# Autodesk Inventor assembly: ASM_Micron_Exploded
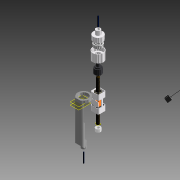
[picture p0: Inventor's stored thumbnail of the model, 180x180]
Saved by Autodesk Inventor 2011 SP2 (Build 150309200, 309)
## iProperties
Created: 2013-06-24
Part Number: ASM_Micron_Exploded
Document SubType Name: Assembly
Designer: sungwook
Author: sungwook
## Documents named in this file (10)
- C:\Users\sungwook\Documents\Inventor\Micron22_top_adj_02082013\06242013_FigGen\ASM_Micron_Motor_Exploded.iam
- C:\Users\sungwook\Documents\Inventor\Micron22_top_adj_02082013\Parts\Motor Units\MU_Motor_Asm_Frame_new3.ipt
- C:\Users\sungwook\Documents\Inventor\Micron22_top_adj_02082013\Parts\Motor Units\Squiggle\MU_SQ_Motor_Base.iam
- C:\Users\sungwook\Documents\Inventor\Micron22_top_adj_02082013\Parts\Motor Units\MU_Motor_Thread.ipt
- C:\Users\sungwook\Documents\Inventor\Micron22_top_adj_02082013\Parts\Motor Units\MU_Bearing_Housing_Inner.ipt
- C:\Users\sungwook\Documents\Inventor\Micron22_top_adj_02082013\Parts\Motor Units\MU_Prolene.ipt
- C:\Users\sungwook\Documents\Inventor\Micron22_top_adj_02082013\Parts\Motor Units\MU_Bottom_Stop.ipt
- C:\Users\sungwook\Documents\Inventor\Micron22_top_adj_02082013\Parts\Motor Units\MU_Bearing(681h).ipt
- C:\Users\sungwook\Documents\Inventor\Micron22_top_adj_02082013\Parts\Motor Units\MU_Motor_Coupling_3.ipt
- C:\Users\sungwook\Documents\Inventor\Micron22_top_adj_02082013\Parts\Motor Units\MU_Bearing_Retainer.ipt
## Components (10 placed, 9 different names)
1. MU_Motor_Asm_Frame_new3:1 — Mate:2, Mate:3, Mate:11
2. MU_SQ_Motor_Base:1 [sub-assembly] — Mate:1, Mate:2, Mate:3, Mate:4
3. MU_Motor_Thread:1 — Mate:1, Mate:5, Mate:10
4. MU_Bearing_Housing_Inner:1 — Mate:8, Mate:9
5. MU_Prolene:1 — Mate:9
6. MU_Prolene:2 — Mate:11
7. MU_Bottom_Stop:1 — Mate:10
8. MU_Bearing(681h):1 — Mate:7, Mate:8
9. MU_Motor_Coupling_3:1 — Mate:5, Mate:6, Mate:7
10. MU_Bearing_Retainer:1 — Mate:6
## Relationships (11: Mate 11)
- Mate:1: MU_SQ_Motor_Base:1 ↔ MU_Motor_Thread:1
- Mate:2: MU_Motor_Asm_Frame_new3:1 ↔ MU_SQ_Motor_Base:1
- Mate:3: MU_Motor_Asm_Frame_new3:1 ↔ MU_SQ_Motor_Base:1
- Mate:4: MU_SQ_Motor_Base:1
- Mate:5: MU_Motor_Thread:1 ↔ MU_Motor_Coupling_3:1
- Mate:6: MU_Motor_Coupling_3:1 ↔ MU_Bearing_Retainer:1
- Mate:7: MU_Bearing(681h):1 ↔ MU_Motor_Coupling_3:1
- Mate:8: MU_Bearing_Housing_Inner:1 ↔ MU_Bearing(681h):1
- Mate:9: MU_Bearing_Housing_Inner:1 ↔ MU_Prolene:1
- Mate:10: MU_Motor_Thread:1 ↔ MU_Bottom_Stop:1
- Mate:11: MU_Motor_Asm_Frame_new3:1 ↔ MU_Prolene:2
